# Autodesk Inventor assembly: yaw-frame
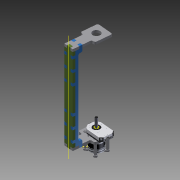
[picture p0: Inventor's stored thumbnail of the model, 180x180]
Saved by Autodesk Inventor 2015 (Build 190159000, 159)
## iProperties
Created: 2015-11-30
Part Number: yaw-frame
Document SubType Name: Assembly
Designer: jufranz
Author: jufranz
## Documents named in this file (9)
- \\engin-labs.m.storage.umich.edu\jufranz\windat.V2\Documents\Inventor\perspection\yaw-frame.iam
- \\engin-labs.m.storage.umich.edu\jufranz\windat.V2\Documents\Inventor\perspection\Imported Components\Tiger-Motor\Tiger-Motor.iam
- \\engin-labs.m.storage.umich.edu\jufranz\windat.V2\Documents\Inventor\perspection\Imported Components\motor_base\motor_base.ipt
- \\engin-labs.m.storage.umich.edu\jufranz\windat.V2\Documents\Inventor\perspection\standoff.ipt
- \\engin-labs.m.storage.umich.edu\jufranz\windat.V2\Documents\Inventor\perspection\pitch_mount.ipt
- \\engin-labs.m.storage.umich.edu\jufranz\windat.V2\Documents\Inventor\perspection\amt102\amt102-v.iam
- \\engin-labs.m.storage.umich.edu\jufranz\windat.V2\Documents\Inventor\perspection\base.ipt
- \\engin-labs.m.storage.umich.edu\jufranz\windat.V2\Documents\Inventor\perspection\base_support.ipt
- \\engin-labs.m.storage.umich.edu\jufranz\windat.V2\Documents\Inventor\perspection\pitch_support.ipt
## Components (12 placed, 8 different names)
1. Tiger-Motor:1 [sub-assembly] — Insert:1, Insert:2
2. motor_base:1 — Insert:1, Insert:2, Insert:3, Insert:4, Insert:5, Insert:6
3. standoff:1 — Insert:6
4. standoff:2 — Insert:4, Insert:8
5. standoff:3 — Insert:5, Insert:7
6. standoff:4 — Insert:3
7. pitch_mount:1 — Insert:7, Insert:8, Insert:9, Mate:1, Mate:2, Mate:3, Mate:4, Mate:5, Mate:6, Mate:7, Mate:8, Mate:9
8. amt102-v:1 [sub-assembly] — Insert:9
9. base:1 — Mate:1, Mate:2, Mate:3, Mate:10
10. base_support:1 — Mate:4, Mate:5, Mate:6, Mate:11
11. base_support:2 — Mate:7, Mate:8, Mate:9, Mate:12
12. pitch_support:1 — Mate:10, Mate:11, Mate:12
## Relationships (21: Mate 12, Insert 9)
- Insert:1: Tiger-Motor:1 ↔ motor_base:1
- Insert:2: Tiger-Motor:1 ↔ motor_base:1
- Insert:3: motor_base:1 ↔ standoff:4
- Insert:4: motor_base:1 ↔ standoff:2
- Insert:5: motor_base:1 ↔ standoff:3
- Insert:6: motor_base:1 ↔ standoff:1
- Insert:7: standoff:3 ↔ pitch_mount:1
- Insert:8: standoff:2 ↔ pitch_mount:1
- Insert:9: pitch_mount:1 ↔ amt102-v:1
- Mate:1: pitch_mount:1 ↔ base:1
- Mate:2: pitch_mount:1 ↔ base:1
- Mate:3: pitch_mount:1 ↔ base:1
- Mate:4: pitch_mount:1 ↔ base_support:1
- Mate:5: pitch_mount:1 ↔ base_support:1
- Mate:6: pitch_mount:1 ↔ base_support:1
- Mate:7: pitch_mount:1 ↔ base_support:2
- Mate:8: pitch_mount:1 ↔ base_support:2
- Mate:9: pitch_mount:1 ↔ base_support:2
- Mate:10: base:1 ↔ pitch_support:1
- Mate:11: base_support:1 ↔ pitch_support:1
- Mate:12: base_support:2 ↔ pitch_support:1
